# Autodesk Inventor assembly: Montagem do Conjunto de Came
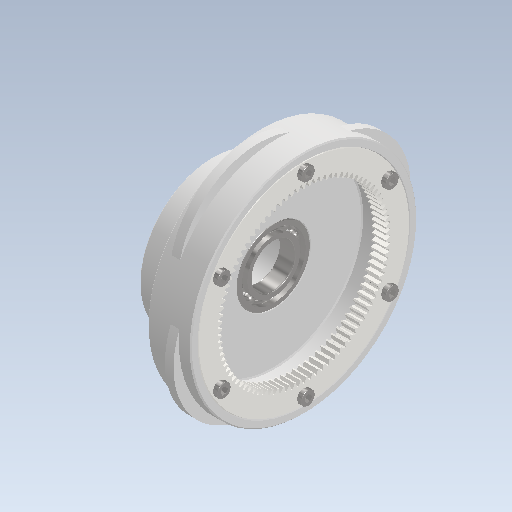
[picture p0: Inventor's stored thumbnail of the model, 512x512]
Saved by Autodesk Inventor 2021 (Build 250183000, 183)
## iProperties
Category: 10
Company: UFABC
Created: 2021-07-26
Document SubType Name: Assembly
Designer: Giovanni
Checked By: Prof. Luis
User Status: 1:4
Description: 01
Author: Giovanni Rodrigues Dias
Title: Montagem do Conjunto de Came
Keywords: 7
Revision Number: 01
## Documents named in this file (9)
- C:\Users\irineu\Documents\Inventor\MotorRadial7\Conjunto de Came.iam
- C:\Users\irineu\Documents\Inventor\MotorRadial7\Peça21.ipt
- C:\Users\irineu\Documents\Inventor\MotorRadial7\Peça23.ipt
- C:\Users\irineu\Documents\Inventor\MotorRadial7\Engrenagens 3.iam
- C:\Users\irineu\Documents\Inventor\Content Center Files\R2021\pt-BR\DIN BEARING(1)\DIN 625 SKF - SKF 6008.ipt
- C:\Users\irineu\Documents\Inventor\MotorRadial7\Peça22.ipt
- C:\Users\irineu\Documents\Inventor\Content Center Files\R2021\pt-BR\DIN 912\DIN 912 - M6 x 1 x 16 x 13,5.ipt
- C:\Users\irineu\Documents\Inventor\Content Center Files\R2021\pt-BR\DIN 912\DIN 912 - M8 x 1,25 x 16 x 12,875.ipt
- C:\Users\irineu\Documents\Inventor\Content Center Files\R2021\pt-BR\DIN 913\DIN 913 - M8 x 12.ipt
## Components (18 placed, 8 different names)
1. Peça21:1 — Inserir:1, Coincidente:2, Coincidente:3, Inserir:2, Inserir:3, Inserir:4, Tangente:1
2. Peça23:1 — Inserir:1, Coincidente:1, Coincidente:6
3. Engrenagens 3:1 [sub-assembly] — Coincidente:2, Coincidente:3, Coincidente:4, Inserir:6
4. DIN 625 SKF SKF 6008:1 — Inserir:2
5. DIN 625 SKF SKF 6008:2 — Inserir:3
6. Peça22:1 — Inserir:4, Coincidente:5, Inserir:5
7. DIN 912 - substituído por DIN EN ISO 4762 M6 x 16:1 — Inserir:5
8. DIN 912 - substituído por DIN EN ISO 4762 M6 x 16:2
9. DIN 912 - substituído por DIN EN ISO 4762 M6 x 16:3
10. DIN 912 - substituído por DIN EN ISO 4762 M6 x 16:4
11. DIN 912 - substituído por DIN EN ISO 4762 M8 x 16:1 — Inserir:6
12. DIN 912 - substituído por DIN EN ISO 4762 M8 x 16:2
13. DIN 912 - substituído por DIN EN ISO 4762 M8 x 16:3
14. DIN 912 - substituído por DIN EN ISO 4762 M8 x 16:4
15. DIN 912 - substituído por DIN EN ISO 4762 M8 x 16:5
16. DIN 912 - substituído por DIN EN ISO 4762 M8 x 16:6
17. DIN 913 M8 x 12:1 — Coincidente:6, Tangente:1
18. DIN 913 M8 x 12:2
## Component patterns: (4 elements, first: DIN 912 - substituído por DIN EN ISO 4762 M6 x 16:1), (6 elements, first: DIN 912 - substituído por DIN EN ISO 4762 M8 x 16:1), (2 elements, first: DIN 913 M8 x 12:1)
## Relationships (13: Insert 6, Mate 6, Tangent 1)
- Inserir:1: Peça21:1 ↔ Peça23:1
- Coincidente:1 [Mate]: Peça23:1
- Coincidente:2 [Mate]: Peça21:1 ↔ Engrenagens 3:1
- Coincidente:3 [Mate]: Peça21:1 ↔ Engrenagens 3:1
- Coincidente:4 [Mate]: Engrenagens 3:1
- Inserir:2: Peça21:1 ↔ DIN 625 SKF SKF 6008:1
- Inserir:3: Peça21:1 ↔ DIN 625 SKF SKF 6008:2
- Inserir:4: Peça21:1 ↔ Peça22:1
- Coincidente:5 [Mate]: Peça22:1
- Inserir:5: Peça22:1 ↔ DIN 912 - substituído por DIN EN ISO 4762 M6 x 16:1
- Inserir:6: Engrenagens 3:1 ↔ DIN 912 - substituído por DIN EN ISO 4762 M8 x 16:1
- Coincidente:6 [Mate]: Peça23:1 ↔ DIN 913 M8 x 12:1
- Tangente:1: Peça21:1 ↔ DIN 913 M8 x 12:1
